# Autodesk Inventor assembly: TestMergerWseat
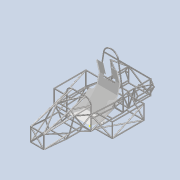
[picture p0: Inventor's stored thumbnail of the model, 180x180]
Saved by Autodesk Inventor 2021 (Build 250183000, 183)
## iProperties
Created: 2020-10-11
Part Number: TestMergerWseat
Document SubType Name: Assembly
Designer: qv17m
Author: qv17m
## Documents named in this file (7)
- D:\PhotonUser\Desktop\FullCarV1.5.2\FullCarV1.5.2\FullCarV1.5.2\FullCarV1.5.iam
- D:\PhotonUser\Desktop\FullCarV1.5.2\FullCarV1.5.2\FullCarV1.5.2\GLV\GLVBattery.ipt
- D:\PhotonUser\Desktop\FullCarV1.5.2\FullCarV1.5.2\FullCarV1.5.2\FullFrame.002\FullFrame.002.iam
- D:\PhotonUser\Desktop\FullCarV1.5.2\FullCarV1.5.2\FullCarV1.5.2\Frame\Seat3DSketch.ipt
- D:\PhotonUser\Desktop\FullCarV1.5.2\FullCarV1.5.2\FullCarV1.5.2\Frame\harness attachments.ipt
- D:\PhotonUser\Desktop\FullCarV1.5.2\FullCarV1.5.2\FullCarV1.5.2\Frame\Seat tabsnew.ipt
- D:\PhotonUser\Desktop\FullCarV1.5.2\FullCarV1.5.2\FullCarV1.5.2\Frame\Seat tab to frame mount.ipt
## Components (11 placed, 6 different names)
1. GLVBattery:1
2. FullFrame.002:1 [sub-assembly] — Mate:3, Mate:5, Mate:6, Mate:7, Mate:8, Mate:9, Mate:10, Mate:11, Angle:1, Angle:2, Angle:3, Angle:4, Angle:5, Angle:6, Mate:18, Mate:19, Angle:7, Mate:20, Angle:8, Mate:21
3. Seat3DSketch:1 — Mate:22, Mate:23, Mate:24, Mate:25
4. harness attachments:3 — Mate:19, Angle:7, Mate:20
5. harness attachments:4 — Mate:18, Angle:8, Mate:21
6. Seat tabsnew:1 — Angle:5, Mate:12, Mate:13, Mate:14, Mate:23, Mate:26
7. Seat tabsnew:2 — Angle:6, Mate:15, Mate:16, Mate:17, Mate:22, Mate:25, Mate:26
8. Seat tab to frame mount:1 — Mate:5, Mate:8, Angle:2, Mate:16, Mate:17
9. Seat tab to frame mount:2 — Mate:3, Mate:9, Angle:4, Mate:12
10. Seat tab to frame mount:3 — Mate:6, Mate:7, Angle:1, Mate:13, Mate:14
11. Seat tab to frame mount:4 — Mate:10, Mate:11, Angle:3, Mate:15
## Relationships (31: Mate 23, Angle 8)
- Mate:3: FullFrame.002:1 ↔ Seat tab to frame mount:2
- Mate:5: FullFrame.002:1 ↔ Seat tab to frame mount:1
- Mate:6: FullFrame.002:1 ↔ Seat tab to frame mount:3
- Mate:7: FullFrame.002:1 ↔ Seat tab to frame mount:3
- Mate:8: FullFrame.002:1 ↔ Seat tab to frame mount:1
- Mate:9: FullFrame.002:1 ↔ Seat tab to frame mount:2
- Mate:10: FullFrame.002:1 ↔ Seat tab to frame mount:4
- Mate:11: FullFrame.002:1 ↔ Seat tab to frame mount:4
- Angle:1 (270 deg): FullFrame.002:1 ↔ Seat tab to frame mount:3
- Angle:2 (270 deg): FullFrame.002:1 ↔ Seat tab to frame mount:1
- Angle:3 (270 deg): FullFrame.002:1 ↔ Seat tab to frame mount:4
- Angle:4 (270 deg): FullFrame.002:1 ↔ Seat tab to frame mount:2
- Angle:5 (0 deg): FullFrame.002:1 ↔ Seat tabsnew:1
- Mate:12: Seat tabsnew:1 ↔ Seat tab to frame mount:2
- Mate:13: Seat tabsnew:1 ↔ Seat tab to frame mount:3
- Mate:14 (6.35 mm): Seat tabsnew:1 ↔ Seat tab to frame mount:3
- Angle:6 (0 deg): FullFrame.002:1 ↔ Seat tabsnew:2
- Mate:15: Seat tabsnew:2 ↔ Seat tab to frame mount:4
- Mate:16: Seat tabsnew:2 ↔ Seat tab to frame mount:1
- Mate:17 (6.35 mm): Seat tabsnew:2 ↔ Seat tab to frame mount:1
- Mate:18: FullFrame.002:1 ↔ harness attachments:4
- Mate:19: FullFrame.002:1 ↔ harness attachments:3
- Angle:7 (0 deg): FullFrame.002:1 ↔ harness attachments:3
- Mate:20: FullFrame.002:1 ↔ harness attachments:3
- Angle:8 (180 deg): FullFrame.002:1 ↔ harness attachments:4
- Mate:21: FullFrame.002:1 ↔ harness attachments:4
- Mate:22: Seat3DSketch:1 ↔ Seat tabsnew:2
- Mate:23: Seat3DSketch:1 ↔ Seat tabsnew:1
- Mate:24 (-238 mm): Seat3DSketch:1
- Mate:25: Seat3DSketch:1 ↔ Seat tabsnew:2
- Mate:26 (25 mm): Seat tabsnew:1 ↔ Seat tabsnew:2
